# Autodesk Inventor assembly: 39172
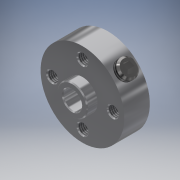
[picture p0: Inventor's stored thumbnail of the model, 180x180]
Saved by Autodesk Inventor 2017.1 (Build 211199000, 199)
## iProperties
Category: Axle Hardware
Company: Autodesk Inc.
Created: 2017-01-02
Part Number: 39172
Document SubType Name: Assembly
Designer: Autodesk Inc.
Catalog Web Link: http://www.tetrixrobotics.com/TETRIX_Axle_Hubs
Vendor: Tetrix
Author: Autodesk Inc.
## Documents named in this file (3)
- D:\FIRST\FTC KOP 2017\FTC 2017 KOP\Tetrix\Tetrix_39172.iam
- D:\FIRST\FTC KOP 2017\FTC 2017 KOP\Tetrix\Tetrix_739172_Collar.ipt
- D:\FIRST\FTC KOP 2017\FTC 2017 KOP\Tetrix\Tetrix_739172_Screw.ipt
## Components (2 placed, 2 different names)
1. Tetrix_39172_Collar:1 — Mate:1
2. Tetrix_39172_Screw:1 — Mate:1
## Relationships (1: Mate 1)
- Mate:1: Tetrix_39172_Collar:1 ↔ Tetrix_39172_Screw:1
